# Autodesk Inventor assembly: radni_sto_final
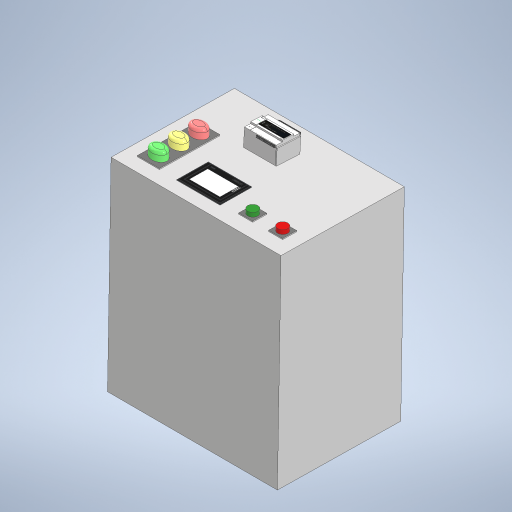
[picture p0: Inventor's stored thumbnail of the model, 512x512]
Saved by Autodesk Inventor 2023 (Build 270158000, 158)
## iProperties
Created: 2022-07-08
Part Number: radni_sto_final
Document SubType Name: Assembly
Designer: User
Author: User
## Documents named in this file (4)
- C:\Users\User\Desktop\PMS\Seminarski rad\Inventor_sheme\radni_sto_final.iam
- C:\Users\User\Desktop\PMS\Seminarski rad\Inventor_sheme\radni_sto.ipt
- C:\Users\User\Desktop\PMS\Seminarski rad\HMI\6av21448gc100aa0.iam
- C:\Users\User\Desktop\PMS\Seminarski rad\Inventor_sheme\PLC.ipt
## Components (3 placed, 3 different names)
1. radni_sto:1 — Mate:1
2. PLC:1
3. 6av21448gc100aa0:2 [sub-assembly] — Mate:1
## Relationships (1: Mate 1)
- Mate:1 (-30 mm): radni_sto:1 ↔ 6av21448gc100aa0:2
